# Autodesk Inventor assembly: link3
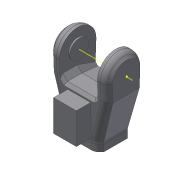
[picture p0: Inventor's stored thumbnail of the model, 180x180]
Saved by Autodesk Inventor 2018 (Build 220112000, 112)
## iProperties
Created: 2019-11-23
Part Number: link3
Document SubType Name: Assembly
Designer: Clevo
Author: Clevo
## Documents named in this file (3)
- E:\RobotArm\Software\URDF_Files\link3.iam
- E:\RobotArm\Software\URDF_Files\link3.ipt
- E:\RobotArm\Software\URDF_Files\link3bearing_carrier.ipt
## Components (2 placed, 2 different names)
1. link3:1 — Flush:1, Flush:2, Mate:1
2. link3bearing_carrier:1 — Flush:1, Flush:2, Mate:1
## Relationships (3: Flush 2, Mate 1)
- Flush:1: link3:1 ↔ link3bearing_carrier:1
- Flush:2: link3:1 ↔ link3bearing_carrier:1
- Mate:1: link3:1 ↔ link3bearing_carrier:1
